# Autodesk Inventor assembly: URLM8
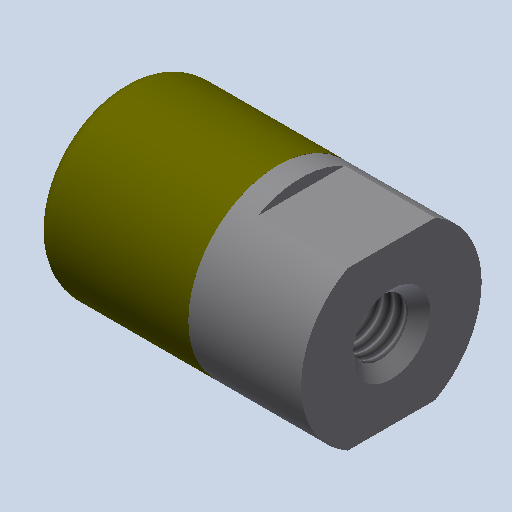
[picture p0: Inventor's stored thumbnail of the model, 512x512]
Saved by Autodesk Inventor 2024.2 (Build 282272000, 272)
## iProperties
Category: PARTsolutions
Company: MISUMI
Created: 2024-01-11
Part Number: URLM8
Description: URLH, URLM, URLL-Urethane Pushers -Tapped - Flat
Vendor: MISUMI
Document SubType Name: Assembly
Designer: psAdmin
Manufacturer: MISUMI
Mass: 0.548413 g
Surface Area: 6.69407 cm^2
Volume: 0.548413 cm^3
Density: 1 g/cm^3
Catalog Web Link: https://jp.misumi-ec.com/vona2/detail/110302358760/?ProductCode=URLM8
PSOL_IDENT_0: {$CADENAS_DATA/23d-libs/misumi/metric/34_cylinders/urlh_asmtab.prj},177 {VTYP=3D},{STYP=ASSTAB},{NB=
PSOL_IDENT_1: URLM8},{LINA=URLM8},{NN=URLH, URLM, URLL},{DATE=04.06.2021 00:06:22},{GEOMDATE=02.09.2014},{VERSION=
PSOL_IDENT_2: },{LINEID=10},{WBVAR=MATP,HARDP,M},{WBNUMERIC=}  {NB=URLM8},{LINA=URLM8},{KT=DUMMY},{PN=URLM8},{TYPE=
PSOL_IDENT_3: URLM},{MATP=2},{MATP1='1', 'Ether Polyurethane', '2', 'Ester Polyurethane'},{HARDP=2},{HARD0='2', 'S
PSOL_IDENT_4: hore A70','3','Shore A50'},{D=8},{L=12},{M=1},{MALG='1','M3x0.5'},{SR1=8},{R2=1.0},{LL1=5},{LL2=4},{
PSOL_IDENT_5: W=7},{NDM=3},{KDM=2.459},{P=0.50},{ALG=},{PPATH=urlh_temp.prj}
NB: URLM8
NN: URLH, URLM, URLL
NT: Urethane Pushers -Tapped - Flat
NBSYN: $PN.
LINA: URLM8
CATALOG: Misumi
PN: URLM8
MATP: Ester Polyurethane
HARDP: Shore A70
D: 8
L: 12
M: M3x0.5
SR1: 8
R2: 1
LL1: 5
LL2: 4
W: 7
SUPPLIER: MISUMI
ARTICLENO: URLM8
BOMINFO: URLM8
CREATOR: CADENAS GmbH
Title: URLM8
Author: Cadenas PARTsolutions
Comments: Urethane Pushers -Tapped - Flat
## Documents named in this file (3)
- C:\Users\masato\OneDrive - Chiba Institute of Technology\CIT Brains\RoboCup2024\Mechanic\SUSTAINA-OP2\NativeFiles\Boby\COTS\MisumiComponents\URLM8.iam
- C:\Users\masato\OneDrive - Chiba Institute of Technology\CIT Brains\RoboCup2024\Mechanic\SUSTAINA-OP2\NativeFiles\Boby\COTS\MisumiComponents\URLM8_p.ipt
- C:\Users\masato\OneDrive - Chiba Institute of Technology\CIT Brains\RoboCup2024\Mechanic\SUSTAINA-OP2\NativeFiles\Boby\COTS\MisumiComponents\URLM8_c.ipt
## Components (2 placed, 2 different names)
1. URLM8_p:1 — pusher_Z@1 <-> core_rod_Z@2
2. URLM8_c:1 — pusher_Z@1 <-> core_rod_Z@2
## Relationships (1: Mate 1)
- pusher_Z@1 <-> core_rod_Z@2 [Mate]: URLM8_p:1 ↔ URLM8_c:1
